# Autodesk Inventor assembly: Bumper Assembly V2
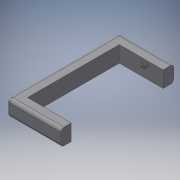
[picture p0: Inventor's stored thumbnail of the model, 180x180]
Saved by Autodesk Inventor 2018 (Build 220112000, 112)
## iProperties
Created: 2020-01-24
Part Number: Bumper Assembly V2
Document SubType Name: Assembly
Designer: S-2512711
Author: S-2512711
## Documents named in this file (3)
- \\studenthome\students\S-2512711\GitHub\2020CAD\Bumpers\Main Assembly File\Bumper Assembly V2.iam
- \\studenthome\students\S-2512711\GitHub\2020CAD\Bumpers\Part Files\Bumper Side V2.ipt
- \\studenthome\students\S-2512711\GitHub\2020CAD\Bumpers\Part Files\Bumper Attachment 1.iam
## Components (2 placed, 2 different names)
1. Bumper Side V2:1 — Mate:1, Mate:2, Mate:3
2. Bumper Attachment 1:1 [sub-assembly] — Mate:1, Mate:2, Mate:3
## Relationships (3: Mate 3)
- Mate:1: Bumper Side V2:1 ↔ Bumper Attachment 1:1
- Mate:2: Bumper Side V2:1 ↔ Bumper Attachment 1:1
- Mate:3: Bumper Side V2:1 ↔ Bumper Attachment 1:1
